# Autodesk Inventor assembly: Chimera Assembly
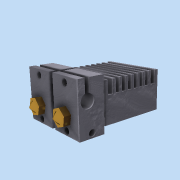
[picture p0: Inventor's stored thumbnail of the model, 180x180]
Saved by Autodesk Inventor 2016 (Build 200138000, 138)
## iProperties
Created: 2016-08-02
Part Number: Chimera Assembly
Document SubType Name: Assembly
Designer: Sam
Author: Sam
## Documents named in this file (7)
- D:\Users\Sam\Documents\Inventor\Zircon3D\Chimera Assembly.iam
- D:\Users\Sam\Documents\Inventor\Zircon3D\Chimera Heatsink.ipt
- D:\Users\Sam\Documents\Inventor\Zircon3D\Chimera Hetsink Brass Insert.ipt
- D:\Users\Sam\Documents\Inventor\Zircon3D\Chimera Heatsink Bowden.ipt
- D:\Users\Sam\Documents\Inventor\Zircon3D\Chimera Heatbreak.ipt
- D:\Users\Sam\Documents\Inventor\Zircon3D\Chimera Heatblock.ipt
- D:\Users\Sam\Documents\Inventor\Zircon3D\Chimera Nozzle.ipt
## Components (11 placed, 6 different names)
1. Chimera Heatsink:1 — Rotational:1, Rotational:2, Rotational:5, Rotational:6
2. Chimera Hetsink Brass Insert:1 — Rotational:1, Rotational:3
3. Chimera Hetsink Brass Insert:2 — Rotational:2, Rotational:4
4. Chimera Heatsink Bowden:1 — Rotational:3
5. Chimera Heatsink Bowden:2 — Rotational:4
6. Chimera Heatbreak:1 — Rotational:5, Rotational:7
7. Chimera Heatbreak:2 — Rotational:6, Rotational:8
8. Chimera Heatblock:1 — Rotational:8, Mate:1
9. Chimera Heatblock:2 — Rotational:7, Mate:2
10. Chimera Nozzle:1 — Mate:1
11. Chimera Nozzle:2 — Mate:2
## Relationships (10: RevoluteJoint 8, Mate 2)
- Rotational:1 [RevoluteJoint]: Chimera Heatsink:1 ↔ Chimera Hetsink Brass Insert:1
- Rotational:2 [RevoluteJoint]: Chimera Heatsink:1 ↔ Chimera Hetsink Brass Insert:2
- Rotational:3 [RevoluteJoint]: Chimera Hetsink Brass Insert:1 ↔ Chimera Heatsink Bowden:1
- Rotational:4 [RevoluteJoint]: Chimera Hetsink Brass Insert:2 ↔ Chimera Heatsink Bowden:2
- Rotational:5 [RevoluteJoint]: Chimera Heatsink:1 ↔ Chimera Heatbreak:1
- Rotational:6 [RevoluteJoint]: Chimera Heatsink:1 ↔ Chimera Heatbreak:2
- Rotational:7 [RevoluteJoint]: Chimera Heatbreak:1 ↔ Chimera Heatblock:2
- Rotational:8 [RevoluteJoint]: Chimera Heatbreak:2 ↔ Chimera Heatblock:1
- Mate:1: Chimera Heatblock:1 ↔ Chimera Nozzle:1
- Mate:2: Chimera Heatblock:2 ↔ Chimera Nozzle:2
